# Autodesk Inventor assembly: Hydraulikzylinder
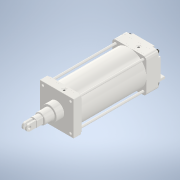
[picture p0: Inventor's stored thumbnail of the model, 180x180]
Saved by Autodesk Inventor 2020.3 (Build 243373000, 373)
## iProperties
Created: 2021-05-29
Part Number: Hydraulikzylinder
Document SubType Name: Assembly
Designer: Preuß P. Ch.
Author: Preuß P. Ch.
## Documents named in this file (9)
- D:\Studium\Praegemaschine\3D-Modelle\Hydraulikzylinder.iam
- C:\Users\user\Documents\Inventor\Hydraulikzylinder\Gehäuse.ipt
- C:\Users\user\Documents\Inventor\Hydraulikzylinder\Deckel_hinten.ipt
- C:\Users\user\Documents\Inventor\Hydraulikzylinder\Gelenkflansch.ipt
- C:\Users\user\Documents\Inventor\Hydraulikzylinder\Kolben.ipt
- C:\Users\user\Documents\Inventor\Hydraulikzylinder\Kolbenstange.ipt
- C:\Users\user\Documents\Inventor\Hydraulikzylinder\Deckel_vorne.ipt
- C:\Users\user\Documents\Inventor\Hydraulikzylinder\Gewindestange.ipt
- C:\Users\user\Documents\Inventor\Content Center Files\R2020\de-DE\ISO 4033(1)\ISO 4033 - M10DIN EN.ipt
## Components (18 placed, 8 different names)
1. Gehäuse:1 — Einfügen:1, Passend:1, Passend:5, Passend:8, Passend:9, Einfügen:9
2. Deckel_hinten:1 — Einfügen:1, Passend:1, Passend:2, Passend:3, Passend:4, Winkel:1, Verfahrweg, Winkel:2
3. Gelenkflansch:1 — Passend:2, Passend:3, Passend:4, Einfügen:2, Einfügen:3, Einfügen:4, Einfügen:5, Einfügen:10, Einfügen:11, Einfügen:12, Einfügen:13
4. Kolben:1 — Passend:5, Passend:6, Passend:7, Verfahrweg, Winkel:2, Unterdrücken_bei_Verfahrweg
5. Kolbenstange:1 — Passend:6, Passend:7, Winkel:1
6. Deckel_vorne:1 — Passend:8, Passend:9, Einfügen:6, Einfügen:7, Einfügen:8, Unterdrücken_bei_Verfahrweg
7. Gewindestange:1 — Einfügen:4
8. Gewindestange:2 — Einfügen:2
9. Gewindestange:3 — Einfügen:3
10. Gewindestange:4 — Einfügen:5
11. DIN EN 24033 M10:1 — Einfügen:6
12. DIN EN 24033 M10:2 — Einfügen:7
13. DIN EN 24033 M10:3 — Einfügen:9
14. DIN EN 24033 M10:4 — Einfügen:8
15. DIN EN 24033 M10:5 — Einfügen:12
16. DIN EN 24033 M10:6 — Einfügen:13
17. DIN EN 24033 M10:7 — Einfügen:11
18. DIN EN 24033 M10:8 — Einfügen:10
## Relationships (26: Insert 13, Mate 11, Angle 2)
- Einfügen:1 [Insert]: Gehäuse:1 ↔ Deckel_hinten:1
- Passend:1 [Mate]: Gehäuse:1 ↔ Deckel_hinten:1
- Passend:2 [Mate]: Deckel_hinten:1 ↔ Gelenkflansch:1
- Passend:3 [Mate]: Deckel_hinten:1 ↔ Gelenkflansch:1
- Passend:4 [Mate]: Deckel_hinten:1 ↔ Gelenkflansch:1
- Passend:5 [Mate]: Gehäuse:1 ↔ Kolben:1
- Passend:6 [Mate]: Kolben:1 ↔ Kolbenstange:1
- Passend:7 [Mate]: Kolben:1 ↔ Kolbenstange:1
- Winkel:1 [Angle] (0 deg): Deckel_hinten:1 ↔ Kolbenstange:1
- Passend:8 [Mate]: Gehäuse:1 ↔ Deckel_vorne:1
- Passend:9 [Mate]: Gehäuse:1 ↔ Deckel_vorne:1
- Verfahrweg [Mate]: Deckel_hinten:1 ↔ Kolben:1
- Einfügen:2 [Insert] (-15 mm): Gelenkflansch:1 ↔ Gewindestange:2
- Einfügen:3 [Insert] (-15 mm): Gelenkflansch:1 ↔ Gewindestange:3
- Einfügen:4 [Insert] (-15 mm): Gelenkflansch:1 ↔ Gewindestange:1
- Einfügen:5 [Insert] (-15 mm): Gelenkflansch:1 ↔ Gewindestange:4
- Winkel:2 [Angle] (0 deg): Deckel_hinten:1 ↔ Kolben:1
- Einfügen:6 [Insert]: Deckel_vorne:1 ↔ DIN EN 24033 M10:1
- Einfügen:7 [Insert]: Deckel_vorne:1 ↔ DIN EN 24033 M10:2
- Einfügen:8 [Insert]: Deckel_vorne:1 ↔ DIN EN 24033 M10:4
- Einfügen:9 [Insert]: Gehäuse:1 ↔ DIN EN 24033 M10:3
- Einfügen:10 [Insert]: Gelenkflansch:1 ↔ DIN EN 24033 M10:8
- Einfügen:11 [Insert]: Gelenkflansch:1 ↔ DIN EN 24033 M10:7
- Einfügen:12 [Insert]: Gelenkflansch:1 ↔ DIN EN 24033 M10:5
- Einfügen:13 [Insert]: Gelenkflansch:1 ↔ DIN EN 24033 M10:6
- Unterdrücken_bei_Verfahrweg [Mate] (228 mm): Kolben:1 ↔ Deckel_vorne:1
